# Autodesk Inventor assembly: monitorControl
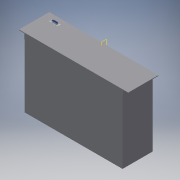
[picture p0: Inventor's stored thumbnail of the model, 180x180]
Saved by Autodesk Inventor 2016 (Build 200138000, 138)
## iProperties
Created: 2016-08-10
Part Number: monitorControl
Document SubType Name: Assembly
Designer: Zara
Author: Zara
## Documents named in this file (3)
- C:\Users\Zara\Documents\hera-cad\Node\monitorControl.iam
- C:\Users\Zara\Documents\hera-cad\Node\monitorControl.ipt
- C:\Users\Zara\Documents\hera-cad\Node\DB15_F.ipt
## Components (2 placed, 2 different names)
1. monitorControl:1 — Mate:1
2. DB15_F:1 — Mate:1
## Relationships (1: Mate 1)
- Mate:1: monitorControl:1 ↔ DB15_F:1
